# Autodesk Inventor assembly: MCARMassembly
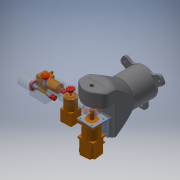
[picture p0: Inventor's stored thumbnail of the model, 180x180]
Saved by Autodesk Inventor 2019 (Build 230136000, 136)
## iProperties
Created: 2019-07-24
Part Number: MCARMassembly
Document SubType Name: Assembly
Designer: Matt
Author: Matt
## Documents named in this file (23)
- C:\Users\Matt\Documents\MAKE\Inventor\Projects\ARM\ARM Models\ARM Assembly\MCARMassembly.iam
- C:\Users\Matt\Documents\MAKE\Inventor\Projects\ARM\ARM Models\ARMparts\BaseCap.ipt
- C:\Users\Matt\Documents\MAKE\Inventor\Projects\ARM\ARM Models\Components\NEMA14wGBX.ipt
- C:\Users\Matt\Documents\MAKE\Inventor\Projects\ARM\ARM Models\ARMparts\BaseMid.ipt
- C:\Users\Matt\Documents\MAKE\Inventor\Projects\ARM\ARM Models\Components\Bearing.ipt
- C:\Users\Matt\Documents\MAKE\Inventor\Projects\ARM\ARM Models\ARMparts\BaseUpper1.ipt
- C:\Users\Matt\Documents\MAKE\Inventor\Projects\ARM\ARM Models\ARMparts\BaseUpper2.ipt
- C:\Users\Matt\Documents\MAKE\Inventor\Projects\ARM\ARM Models\Components\NEMA23wGBX.ipt
- C:\Users\Matt\Documents\MAKE\Inventor\Projects\ARM\ARM Models\Components\NEMA23MotorMount.ipt
- C:\Users\Matt\Documents\MAKE\Inventor\Projects\ARM\ARM Models\Components\14mm key hub.ipt
- C:\Users\Matt\Documents\MAKE\Inventor\Projects\ARM\ARM Models\ARMparts\Arm1.ipt
- C:\Users\Matt\Documents\MAKE\Inventor\Projects\ARM\ARM Models\Components\NEMA17wGBX.ipt
- C:\Users\Matt\Documents\MAKE\Inventor\Projects\ARM\ARM Models\Components\8mm hub.ipt
- C:\Users\Matt\Documents\MAKE\Inventor\Projects\ARM\ARM Models\Components\Roller Chain Sprocket 8mm.ipt
- C:\Users\Matt\Documents\MAKE\Inventor\Projects\ARM\ARM Models\Components\8mm Roller Bearing.ipt
- C:\Users\Matt\Documents\MAKE\Inventor\Projects\ARM\ARM Models\ARMparts\Arm2A.ipt
- C:\Users\Matt\Documents\MAKE\Inventor\Projects\ARM\ARM Models\Components\12mm thrust bearing.ipt
- C:\Users\Matt\Documents\MAKE\Inventor\Projects\ARM\ARM Models\Components\8mm rod.ipt
- C:\Users\Matt\Documents\MAKE\Inventor\Projects\ARM\ARM Models\Components\8mm rod2.ipt
- C:\Users\Matt\Documents\MAKE\Inventor\Projects\ARM\ARM Models\Components\6mm belt pulley.ipt
- C:\Users\Matt\Documents\MAKE\Inventor\Projects\ARM\ARM Models\Components\8mm belt pulley.ipt
- C:\Users\Matt\Documents\MAKE\Inventor\Projects\ARM\ARM Models\Components\8mm thrust bearing.ipt
- C:\Users\Matt\Documents\MAKE\Inventor\Projects\ARM\ARM Models\ARMparts\Arm2B.ipt
## Components (30 placed, 22 different names)
1. NEMA14wGBX:1 — Rigid:1, Rotational:3
2. BaseCap:1 — Cylindrical:3
3. BaseMid:1 — Rigid:1, Rotational:2, Cylindrical:3
4. Bearing:1 — Rotational:2
5. BaseUpper1:1 — Rotational:3, Rotational:4
6. BaseUpper2:1 — Rotational:4, Rotational:7, Rotational:8
7. Arm1:1 — Rotational:7, Rotational:9, Rotational:11, Rotational:13, Rotational:17, Rotational:18
8. 14mm key hub:2 — Rotational:9
9. NEMA23MotorMount:1 — Rotational:8, Rotational:10
10. NEMA17wGBX:1 — Rotational:11, Cylindrical:8
11. NEMA23wGBX:1 — Rotational:10
12. Roller Chain Sprocket 8mm:1 — Cylindrical:8
13. Roller Chain Sprocket 8mm:2 — Rotational:19
14. 8mm Roller Bearing:1 — Rotational:13, Rotational:14
15. 8mm Roller Bearing:2 — Rotational:17
16. 8mm hub:1 — Rotational:12
17. Arm2A:1 — Rotational:12, Rigid:2, Rotational:20, Rotational:21, Rotational:22, Rotational:23, Rotational:24, Rotational:25
18. 12mm thrust bearing:1 — Rotational:14, Rotational:20
19. 12mm thrust bearing:2 — Rotational:18, Rotational:19
20. 8mm rod:1 — Rigid:2
21. NEMA14wGBX:2 — Rotational:21, Rigid:3
22. 8mm rod2:1 — Rigid:4, Cylindrical:9
23. 6mm belt pulley:1 — Rigid:3
24. 8mm belt pulley:1 — Rigid:4, Rigid:5
25. 8mm thrust bearing:1 — Rotational:24, Rigid:5
26. 8mm thrust bearing:2 — Rotational:25
27. 8mm Roller Bearing:3 — Rotational:23
28. 8mm Roller Bearing:4 — Rotational:22
29. Arm2B:1 — Rotational:26
30. 8mm hub:2 — Rotational:26, Cylindrical:9
## Relationships (29: RevoluteJoint 21, WeldJoint 5, CylindricalJoint 3)
- Rigid:1 [WeldJoint]: NEMA14wGBX:1 ↔ BaseMid:1
- Rotational:2 [RevoluteJoint]: BaseMid:1 ↔ Bearing:1
- Rotational:3 [RevoluteJoint]: NEMA14wGBX:1 ↔ BaseUpper1:1
- Cylindrical:3: BaseCap:1 ↔ BaseMid:1
- Rotational:4 [RevoluteJoint]: BaseUpper1:1 ↔ BaseUpper2:1
- Rotational:7 [RevoluteJoint] (3 mm): BaseUpper2:1 ↔ Arm1:1
- Rotational:8 [RevoluteJoint]: BaseUpper2:1 ↔ NEMA23MotorMount:1
- Rotational:9 [RevoluteJoint]: Arm1:1 ↔ 14mm key hub:2
- Rotational:10 [RevoluteJoint]: NEMA23MotorMount:1 ↔ NEMA23wGBX:1
- Rotational:11 [RevoluteJoint]: Arm1:1 ↔ NEMA17wGBX:1
- Cylindrical:8: NEMA17wGBX:1 ↔ Roller Chain Sprocket 8mm:1
- Rotational:12 [RevoluteJoint]: 8mm hub:1 ↔ Arm2A:1
- Rotational:13 [RevoluteJoint]: Arm1:1 ↔ 8mm Roller Bearing:1
- Rotational:14 [RevoluteJoint] (1.5 mm): 8mm Roller Bearing:1 ↔ 12mm thrust bearing:1
- Rotational:17 [RevoluteJoint]: Arm1:1 ↔ 8mm Roller Bearing:2
- Rotational:18 [RevoluteJoint]: Arm1:1 ↔ 12mm thrust bearing:2
- Rotational:19 [RevoluteJoint]: Roller Chain Sprocket 8mm:2 ↔ 12mm thrust bearing:2
- Rigid:2 [WeldJoint]: Arm2A:1 ↔ 8mm rod:1
- Rotational:20 [RevoluteJoint] (5 mm): Arm2A:1 ↔ 12mm thrust bearing:1
- Rotational:21 [RevoluteJoint]: Arm2A:1 ↔ NEMA14wGBX:2
- Rigid:3 [WeldJoint] (-8 mm): NEMA14wGBX:2 ↔ 6mm belt pulley:1
- Rotational:22 [RevoluteJoint]: Arm2A:1 ↔ 8mm Roller Bearing:4
- Rotational:23 [RevoluteJoint]: Arm2A:1 ↔ 8mm Roller Bearing:3
- Rotational:24 [RevoluteJoint]: Arm2A:1 ↔ 8mm thrust bearing:1
- Rotational:25 [RevoluteJoint]: Arm2A:1 ↔ 8mm thrust bearing:2
- Rigid:4 [WeldJoint]: 8mm rod2:1 ↔ 8mm belt pulley:1
- Rigid:5 [WeldJoint]: 8mm belt pulley:1 ↔ 8mm thrust bearing:1
- Rotational:26 [RevoluteJoint]: Arm2B:1 ↔ 8mm hub:2
- Cylindrical:9: 8mm rod2:1 ↔ 8mm hub:2
